# Autodesk Inventor assembly: Сборка_столбик_зад
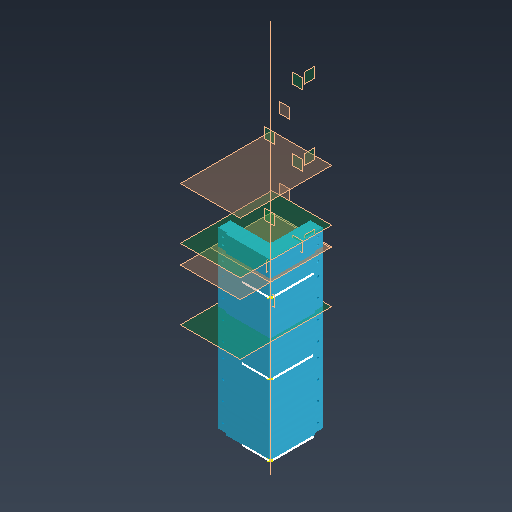
[picture p0: Inventor's stored thumbnail of the model, 512x512]
Saved by Autodesk Inventor 2023.2 (Build 272271030, 271C)
## iProperties
Created: 2025-05-05
Part Number: Сборка_столбик_зад
Document SubType Name: Assembly
Designer: Олег Коноваленко
Author: Олег Коноваленко
## Documents named in this file (3)
- D:\!Rover\Rover\Rover_construction\Сборка_столбик_зад.iam
- D:\!Rover\Rover\Rover_construction\Столбик.ipt
- D:\!Rover\Rover\Rover_construction\Столбик(задний верх).ipt
## Components (3 placed, 2 different names)
1. Столбик:2 — Совмещение:1, Заподлицо:1, Заподлицо:2
2. Столбик:3 — Совмещение:1, Заподлицо:1, Заподлицо:2, Совмещение:2, Заподлицо:3, Заподлицо:4
3. Столбик(задний верх):1 — Совмещение:2, Заподлицо:3, Заподлицо:4
## Relationships (6: Flush 4, Mate 2)
- Совмещение:1 [Mate]: Столбик:2 ↔ Столбик:3
- Заподлицо:1 [Flush]: Столбик:2 ↔ Столбик:3
- Заподлицо:2 [Flush]: Столбик:2 ↔ Столбик:3
- Совмещение:2 [Mate]: Столбик:3 ↔ Столбик(задний верх):1
- Заподлицо:3 [Flush]: Столбик:3 ↔ Столбик(задний верх):1
- Заподлицо:4 [Flush]: Столбик:3 ↔ Столбик(задний верх):1
